# Autodesk Inventor assembly: The Magician's Assistant
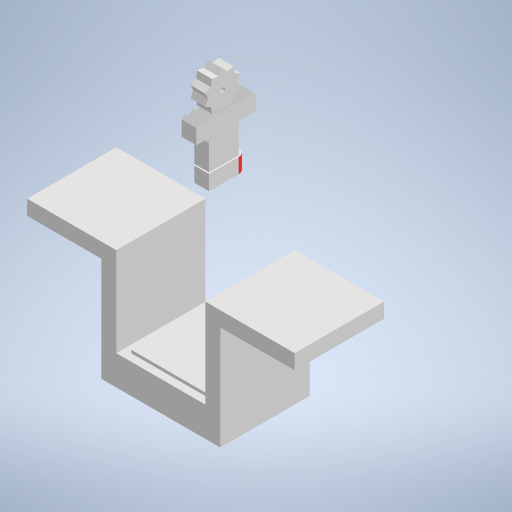
[picture p0: Inventor's stored thumbnail of the model, 512x512]
Saved by Autodesk Inventor 2023 (Build 270158000, 158)
## iProperties
Created: 2023-09-27
Part Number: The Magician's Assistant
Document SubType Name: Assembly
Designer: Turnt
Author: Turnt
## Documents named in this file (6)
- D:\School\ENEE408A\Modeling\The Magician's Assistant.iam
- D:\School\ENEE408A\Modeling\Chassis.ipt
- D:\School\ENEE408A\Modeling\Finger Servo.ipt
- D:\School\ENEE408A\Modeling\Finger.ipt
- D:\School\ENEE408A\Modeling\Finger Rack.ipt
- D:\School\ENEE408A\Modeling\Finger Pinion.ipt
## Components (5 placed, 5 different names)
1. Chassis:1
2. Finger Servo:1 — Rotational:1, Rigid:1
3. Finger:1 — Rotational:1
4. Finger Rack:1 — Rigid:1
5. Finger Pinion:1
## Relationships (2: RevoluteJoint 1, WeldJoint 1)
- Rotational:1 [RevoluteJoint] (2.54 mm): Finger Servo:1 ↔ Finger:1
- Rigid:1 [WeldJoint]: Finger Servo:1 ↔ Finger Rack:1
